# Autodesk Inventor assembly: leg
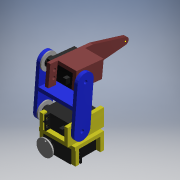
[picture p0: Inventor's stored thumbnail of the model, 180x180]
Saved by Autodesk Inventor 2017 (Build 210142000, 142)
## iProperties
Part Number: leg
Document SubType Name: Assembly
Designer: Alexander Miller
Author: Alexander Miller
## Documents named in this file (5)
- D:\Daten\Documents\Git\Hexapod\3DParts\leg.iam
- D:\Daten\Documents\Git\Hexapod\3DParts\Serov_with_arm.iam
- D:\Daten\Documents\Git\Hexapod\3DParts\Upper_leg.ipt
- D:\Daten\Documents\Git\Hexapod\3DParts\Middle_leg.ipt
- D:\Daten\Documents\Git\Hexapod\3DParts\Lower_leg.ipt
## Components (8 placed, 4 different names)
1. Serov_with_arm:1 [sub-assembly] — Rigid:1, Rotational:1
2. Serov_with_arm:2 [sub-assembly] — Rigid:2
3. Upper_leg:1 — Rigid:1, Rigid:3
4. Upper_leg:2 — Rigid:2, Rigid:3
5. Middle_leg:1 — Rotational:1, Rigid:4
6. Middle_leg:2 — Rigid:4, Rigid:5
7. Serov_with_arm:3 [sub-assembly] — Rigid:5, Rigid:6
8. Lower_leg:1 — Rigid:6
## Relationships (7: WeldJoint 6, RevoluteJoint 1)
- Rigid:1 [WeldJoint]: Serov_with_arm:1 ↔ Upper_leg:1
- Rigid:2 [WeldJoint]: Serov_with_arm:2 ↔ Upper_leg:2
- Rigid:3 [WeldJoint]: Upper_leg:1 ↔ Upper_leg:2
- Rotational:1 [RevoluteJoint]: Serov_with_arm:1 ↔ Middle_leg:1
- Rigid:4 [WeldJoint]: Middle_leg:1 ↔ Middle_leg:2
- Rigid:5 [WeldJoint]: Middle_leg:2 ↔ Serov_with_arm:3
- Rigid:6 [WeldJoint]: Serov_with_arm:3 ↔ Lower_leg:1
